# Autodesk Inventor assembly: 6P Sprocket
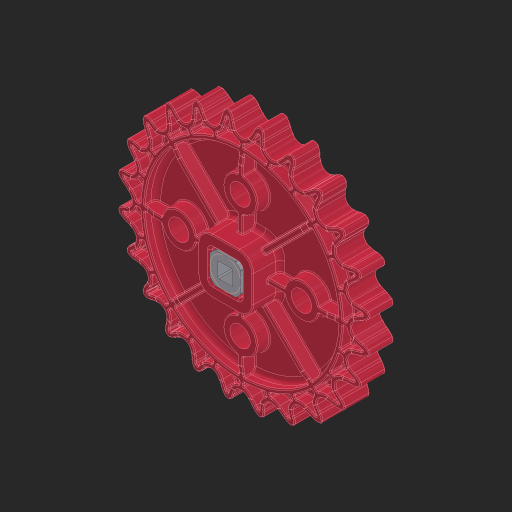
[picture p0: Inventor's stored thumbnail of the model, 512x512]
Saved by Autodesk Inventor 2023 (Build 270158000, 158)
## iProperties
Created: 2022-08-02
Part Number: 6P Sprocket
Document SubType Name: Assembly
Designer: ylu12
Author: ylu12
## Documents named in this file (4)
- C:\Users\ylu12\Documents\GitHub\VEX-CAD-Inventor\Motion\Sprockets\6P Sprocket\6P 24T Sprocket, Square.iam
- C:\Users\ylu12\Documents\GitHub\VEX-CAD-Inventor\Motion\HS Shaft Adapter Square.ipt
- C:\Users\ylu12\Documents\GitHub\VEX-CAD-Inventor\Motion\Sprockets\Reference Files\6P 24T Sprocket.ipt
- C:\Users\ylu12\Documents\GitHub\VEX-CAD-Inventor\Motion\Sprockets\6P Sprocket.iam
## Components (2 placed, 2 different names)
1. Square — Flush:2, Mate:2, Mate:4
2. 24T — Flush:5, Mate:9, Mate:10
## Relationships (6: Mate 4, Flush 2)
- Flush:2 (6.35 mm): Square
- Mate:2: Square
- Mate:4: Square
- Flush:5: 24T
- Mate:9: 24T
- Mate:10: 24T
